# Autodesk Inventor assembly: CuttingLayout
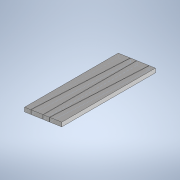
[picture p0: Inventor's stored thumbnail of the model, 180x180]
Saved by Autodesk Inventor 2022 (Build 260153000, 153)
## iProperties
Created: 2021-12-19
Part Number: CuttingLayout
Document SubType Name: Assembly
Designer: dangl
Author: dangl
## Documents named in this file (2)
- C:\Users\dangl\Documents\WoodWork\FloatingBarChair\CuttingLayout.iam
- C:\Users\dangl\Documents\WoodWork\FloatingBarChair\Leg.ipt
## Components (4 placed, 1 different names)
1. Leg:1 — Mate:1, Mate:2, Mate:3, Flush:1, Flush:2, Flush:3, Flush:4, Flush:5, Flush:6
2. Leg:2 — Mate:3, Flush:3, Mate:4, Flush:4
3. Leg:3 — Flush:2, Mate:5, Flush:5
4. Leg:4 — Flush:1, Mate:4, Mate:5, Flush:6
## Relationships (11: Flush 6, Mate 5)
- Mate:1: Leg:1
- Mate:2: Leg:1
- Mate:3 (0.125 mm): Leg:1 ↔ Leg:2
- Flush:1: Leg:1 ↔ Leg:4
- Flush:2: Leg:1 ↔ Leg:3
- Flush:3: Leg:1 ↔ Leg:2
- Mate:4 (0.125 mm): Leg:2 ↔ Leg:4
- Mate:5 (0.125 mm): Leg:3 ↔ Leg:4
- Flush:4: Leg:1 ↔ Leg:2
- Flush:5: Leg:1 ↔ Leg:3
- Flush:6: Leg:1 ↔ Leg:4
